# Autodesk Inventor assembly: Recycling_Hopper
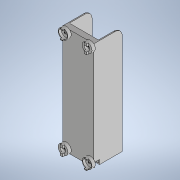
[picture p0: Inventor's stored thumbnail of the model, 180x180]
Saved by Autodesk Inventor 2022 (Build 260153000, 153)
## iProperties
Created: 2022-01-17
Part Number: Recycling_Hopper
Document SubType Name: Assembly
Designer: Work
Author: Work
## Documents named in this file (6)
- C:\Users\Work\Desktop\NewHopper\Recycling_Hopper.iam
- C:\Users\Work\Desktop\NewHopper\Hopper.ipt
- C:\Users\Work\Desktop\DSW\Wk-1\_Resources\Project 3 Autodesk Inventor Files\2. Hopper Assembly\magnet_spacer1V1.ipt
- C:\Users\Work\Desktop\DSW\Wk-1\_Resources\Project 3 Autodesk Inventor Files\2. Hopper Assembly\magneticslot2V1.ipt
- C:\Users\Work\Desktop\DSW\Wk-1\_Resources\Project 3 Autodesk Inventor Files\2. Hopper Assembly\M4 x 16mm Machine Screw.ipt
- C:\Users\Work\Desktop\DSW\Wk-1\_Resources\Project 3 Autodesk Inventor Files\2. Hopper Assembly\M4 Nut.ipt
## Components (13 placed, 5 different names)
1. Hopper:1 — Insert:5, Insert:6, Insert:7, Insert:8, Mate:1, Mate:2, Mate:3, Mate:4, Mate:5, Mate:6, Mate:7, Mate:8, Angle:1, Angle:2, Angle:3, Angle:4
2. M4 x 16mm Machine Screw:1 — Insert:11
3. M4 Nut:1 — Insert:6
4. M4 x 16mm Machine Screw:2 — Insert:12
5. M4 x 16mm Machine Screw:3 — Insert:9
6. M4 x 16mm Machine Screw:4 — Insert:10
7. M4 Nut:2 — Insert:7
8. M4 Nut:3 — Insert:8
9. M4 Nut:4 — Insert:5
10. magneticslot2V1:2 — Mate:4, Mate:6, Angle:4, Insert:10
11. magnet_spacer1V1:2 — Mate:3, Mate:5, Angle:3, Insert:9
12. magneticslot2V1:3 — Mate:2, Mate:7, Angle:1, Insert:11
13. magnet_spacer1V1:3 — Mate:1, Mate:8, Angle:2, Insert:12
## Relationships (20: Insert 8, Mate 8, Angle 4)
- Insert:5: Hopper:1 ↔ M4 Nut:4
- Insert:6: Hopper:1 ↔ M4 Nut:1
- Insert:7: Hopper:1 ↔ M4 Nut:2
- Insert:8: Hopper:1 ↔ M4 Nut:3
- Mate:1: Hopper:1 ↔ magnet_spacer1V1:3
- Mate:2: Hopper:1 ↔ magneticslot2V1:3
- Mate:3: Hopper:1 ↔ magnet_spacer1V1:2
- Mate:4: Hopper:1 ↔ magneticslot2V1:2
- Mate:5: Hopper:1 ↔ magnet_spacer1V1:2
- Mate:6: Hopper:1 ↔ magneticslot2V1:2
- Mate:7: Hopper:1 ↔ magneticslot2V1:3
- Mate:8: Hopper:1 ↔ magnet_spacer1V1:3
- Angle:1 (0 deg): Hopper:1 ↔ magneticslot2V1:3
- Angle:2 (0 deg): Hopper:1 ↔ magnet_spacer1V1:3
- Angle:3 (0 deg): Hopper:1 ↔ magnet_spacer1V1:2
- Angle:4 (0 deg): Hopper:1 ↔ magneticslot2V1:2
- Insert:9: M4 x 16mm Machine Screw:3 ↔ magnet_spacer1V1:2
- Insert:10: M4 x 16mm Machine Screw:4 ↔ magneticslot2V1:2
- Insert:11: M4 x 16mm Machine Screw:1 ↔ magneticslot2V1:3
- Insert:12: M4 x 16mm Machine Screw:2 ↔ magnet_spacer1V1:3
